# Autodesk Inventor assembly: TENSION THREAD
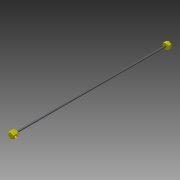
[picture p0: Inventor's stored thumbnail of the model, 180x180]
Saved by Autodesk Inventor 2013 (Build 170138000, 138)
## iProperties
Created: 2013-12-08
Part Number: TENSION THREAD
Document SubType Name: Assembly
Designer: employee
Author: employee
## Documents named in this file (5)
- C:\Users\employee\Desktop\ConceptFORGE\ConceptFORGE\LISA Simpson\INVENTOR FILES\TENSION THREAD.iam
- C:\Users\employee\Desktop\ConceptFORGE\ConceptFORGE\LISA Simpson\INVENTOR FILES\bottom nut.ipt
- C:\Users\employee\Desktop\ConceptFORGE\ConceptFORGE\LISA Simpson\INVENTOR FILES\top nut.ipt
- C:\Users\employee\Desktop\ConceptFORGE\ConceptFORGE\LISA Simpson\INVENTOR FILES\M8 TENSION THREAD.ipt
- C:\Users\employee\Desktop\ConceptFORGE\ConceptFORGE\LISA Simpson\INVENTOR FILES\M8 NUT.ipt
## Components (5 placed, 4 different names)
1. bottom nut:1 — Insert:1, Mate:1, Mate:2, Insert:2, Angle:2
2. top nut:1 — Insert:1, Insert:3, Angle:1
3. M8 TENSION THREAD:1 — Mate:1, Mate:2
4. M8 NUT:1 — Insert:2, Angle:2
5. M8 NUT:2 — Insert:3, Angle:1
## Relationships (7: Insert 3, Mate 2, Angle 2)
- Insert:1 (672.5 mm): bottom nut:1 ↔ top nut:1
- Mate:1: bottom nut:1 ↔ M8 TENSION THREAD:1
- Mate:2: bottom nut:1 ↔ M8 TENSION THREAD:1
- Insert:2: bottom nut:1 ↔ M8 NUT:1
- Insert:3: top nut:1 ↔ M8 NUT:2
- Angle:1 (0 deg): top nut:1 ↔ M8 NUT:2
- Angle:2 (0 deg): bottom nut:1 ↔ M8 NUT:1
